# Autodesk Inventor assembly: SOIC-08 one side
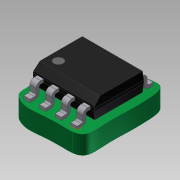
[picture p0: Inventor's stored thumbnail of the model, 180x180]
Saved by Autodesk Inventor 2011 (Build 150239000, 239)
## iProperties
Created: 2010-12-28
Part Number: SOIC-08 one side
Document SubType Name: Assembly
Designer: abbath
Author: abbath
## Documents named in this file (3)
- D:\Abbath\Work\11.2\Сумматор light\КД\RSXX к сумматору\Установка элементов\SOIC-08 установка.iam
- D:\Abbath\Work\11.2\Сумматор light\КД\RSXX к сумматору\Установка элементов\SOIC-08.ipt
- D:\Abbath\Work\11.2\Сумматор light\КД\RSXX к сумматору\Установка элементов\SOIC-08 плата.ipt
## Components (2 placed, 2 different names)
1. SOIC-08:1 — Заподлицо:1
2. SOIC-08 плата:1 — Заподлицо:1
## Relationships (1: Flush 1)
- Заподлицо:1 [Flush]: SOIC-08:1 ↔ SOIC-08 плата:1
